# Autodesk Inventor assembly: 15inOwl
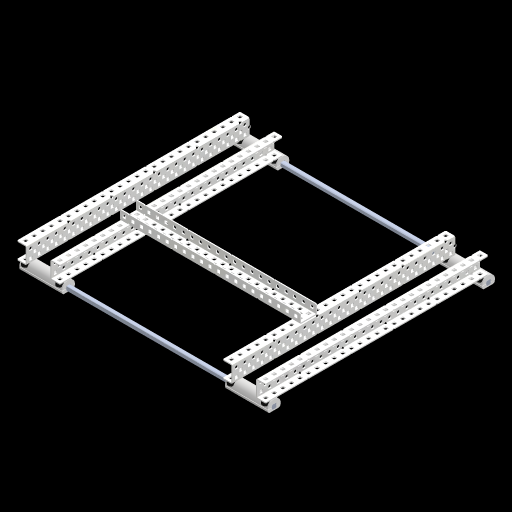
[picture p0: Inventor's stored thumbnail of the model, 512x512]
Saved by Autodesk Inventor 2024.1 (Build 281209000, 209)
## iProperties
Created: 2025-01-28
Part Number: 15inOwl
Document SubType Name: Assembly
Designer: Teddy
Author: Teddy
## Documents named in this file (8)
- C:\Users\Teddy\OneDrive\Desktop\VEX-CAD-Inventor-1.4.0\2024-25 VexGame\15inBotAub\15inOwl.iam
- C:\Users\Teddy\OneDrive\Desktop\VEX-CAD-Inventor-1.4.0\Structure\C Channel\Aluminum 1x2x1\Alu C 1x2x1x21.ipt
- C:\Users\Teddy\OneDrive\Desktop\VEX-CAD-Inventor-1.4.0\Structure\C Channel\Aluminum 1x2x1\Alu C 1x2x1x26.ipt
- C:\Users\Teddy\OneDrive\Desktop\AxleBar.ipt
- C:\Users\Teddy\OneDrive\Desktop\VEX-CAD-Inventor-1.4.0\Motion\Spacers\Spacer Nylon .375 OD\NSpacer .375 OD x .250.ipt
- C:\Users\Teddy\OneDrive\Desktop\VEX-CAD-Inventor-1.4.0\Motion\Spacers\Spacer Nylon .375 OD.ipt
- C:\Users\Teddy\OneDrive\Desktop\VEX-CAD-Inventor-1.4.0\Motion\Shaft HS\Shaft HS\Shaft HS 14.5 in.ipt
- C:\Users\Teddy\OneDrive\Desktop\VEX-CAD-Inventor-1.4.0\Motion\Shaft HS\Shaft HS.ipt
## Components (19 placed, 5 different names)
1. Alu C 1x2x1x21:1 — Insert:1, Insert:2, Insert:3, Insert:4
2. Alu C 1x2x1x26:1 — Insert:3, Insert:4, Insert:17, Insert:20
3. Alu C 1x2x1x26:2 — Insert:1, Insert:2, Insert:13, Insert:16
4. Alu C 1x2x1x26:3 — Insert:14, Insert:15
5. Alu C 1x2x1x26:4 — Insert:18, Insert:19
6. AxleBar:1 — Insert:9, Insert:10, Insert:22
7. AxleBar:2 — Insert:11, Insert:12, Insert:21
8. AxleBar:3 — Insert:7, Insert:8, Insert:23
9. AxleBar:4 — Insert:5, Insert:6, Insert:24
10. NSpacer .375 OD x .250:1 — Insert:5, Insert:18
11. NSpacer .375 OD x .250:2 — Insert:6, Insert:17
12. NSpacer .375 OD x .250:3 — Insert:7, Insert:16
13. NSpacer .375 OD x .250:4 — Insert:8, Insert:15
14. NSpacer .375 OD x .250:5 — Insert:12, Insert:14
15. NSpacer .375 OD x .250:6 — Insert:11, Insert:13
16. NSpacer .375 OD x .250:7 — Insert:10, Insert:20
17. NSpacer .375 OD x .250:8 — Insert:9, Insert:19
18. Shaft HS 14.5 in:1 — Insert:21, Insert:22
19. Shaft HS 14.5 in:2 — Insert:23, Insert:24
## Relationships (24: Insert 24)
- Insert:1: Alu C 1x2x1x21:1 ↔ Alu C 1x2x1x26:2
- Insert:2: Alu C 1x2x1x21:1 ↔ Alu C 1x2x1x26:2
- Insert:3: Alu C 1x2x1x21:1 ↔ Alu C 1x2x1x26:1
- Insert:4: Alu C 1x2x1x21:1 ↔ Alu C 1x2x1x26:1
- Insert:5: AxleBar:4 ↔ NSpacer .375 OD x .250:1
- Insert:6: AxleBar:4 ↔ NSpacer .375 OD x .250:2
- Insert:7: AxleBar:3 ↔ NSpacer .375 OD x .250:3
- Insert:8: AxleBar:3 ↔ NSpacer .375 OD x .250:4
- Insert:9: AxleBar:1 ↔ NSpacer .375 OD x .250:8
- Insert:10: AxleBar:1 ↔ NSpacer .375 OD x .250:7
- Insert:11: AxleBar:2 ↔ NSpacer .375 OD x .250:6
- Insert:12: AxleBar:2 ↔ NSpacer .375 OD x .250:5
- Insert:13: Alu C 1x2x1x26:2 ↔ NSpacer .375 OD x .250:6
- Insert:14: Alu C 1x2x1x26:3 ↔ NSpacer .375 OD x .250:5
- Insert:15: Alu C 1x2x1x26:3 ↔ NSpacer .375 OD x .250:4
- Insert:16: Alu C 1x2x1x26:2 ↔ NSpacer .375 OD x .250:3
- Insert:17: Alu C 1x2x1x26:1 ↔ NSpacer .375 OD x .250:2
- Insert:18: Alu C 1x2x1x26:4 ↔ NSpacer .375 OD x .250:1
- Insert:19: Alu C 1x2x1x26:4 ↔ NSpacer .375 OD x .250:8
- Insert:20: Alu C 1x2x1x26:1 ↔ NSpacer .375 OD x .250:7
- Insert:21: AxleBar:2 ↔ Shaft HS 14.5 in:1
- Insert:22: AxleBar:1 ↔ Shaft HS 14.5 in:1
- Insert:23: AxleBar:3 ↔ Shaft HS 14.5 in:2
- Insert:24: AxleBar:4 ↔ Shaft HS 14.5 in:2
